# Autodesk Inventor assembly: 2 door
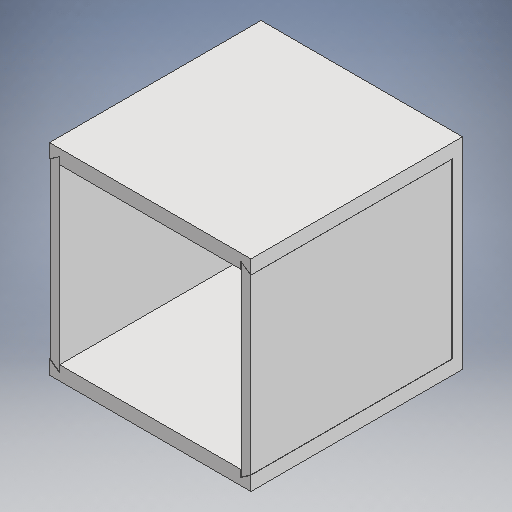
[picture p0: Inventor's stored thumbnail of the model, 512x512]
Saved by Autodesk Inventor 2025.2 (Build 292293000, 293)
## iProperties
Created: 2025-02-23
Part Number: 2 door
Document SubType Name: Assembly
Designer: Alex
Author: Alex
## Documents named in this file (3)
- C:\Shared\alex-bartella-schoolwork\4b03\dr2\2 door.iam
- C:\Shared\alex-bartella-schoolwork\4b03\dr2\main.ipt
- C:\Shared\alex-bartella-schoolwork\4b03\dr2\door.ipt
## Components (3 placed, 2 different names)
1. main:1 — Flush:2, Mate:1, Mate:2, Flush:3, Mate:3, Flush:4
2. door:1 — Flush:2, Mate:1, Mate:2
3. door:2 — Flush:3, Mate:3, Flush:4
## Relationships (6: Flush 3, Mate 3)
- Flush:2 (0.1 mm): main:1 ↔ door:1
- Mate:1 (0.1 mm): main:1 ↔ door:1
- Mate:2: main:1 ↔ door:1
- Flush:3 (0.1 mm): main:1 ↔ door:2
- Mate:3 (0.1 mm): main:1 ↔ door:2
- Flush:4: main:1 ↔ door:2
